# Autodesk Inventor assembly: caly_stół
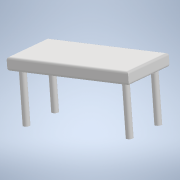
[picture p0: Inventor's stored thumbnail of the model, 180x180]
Saved by Autodesk Inventor 2021 (Build 250183000, 183)
## iProperties
Created: 2020-04-11
Part Number: caly_stół
Document SubType Name: Assembly
Designer: dyrag
Author: dyrag
## Documents named in this file (3)
- C:\Users\dyrag\Desktop\Projects\AutoCAD_Inventor_projects\stół\caly_stół.iam
- C:\Users\dyrag\Desktop\Projects\AutoCAD_Inventor_projects\stół\blat.ipt
- C:\Users\dyrag\Desktop\Projects\AutoCAD_Inventor_projects\stół\Noga.ipt
## Components (6 placed, 2 different names)
1. blat:1 — Zestawiające:1, Zestawiające:2, Zestawiające:3, Zestawiające:4, Równoległe:1, Równoległe:2, Zestawiające:5, Zestawiające:6, Zestawiające:7, Równoległe:3, Równoległe:4, Zestawiające:8, Równoległe:5, Równoległe:6, Zestawiające:9, Równoległe:7, Równoległe:8
2. Noga:1 — Zestawiające:4, Równoległe:1, Równoległe:2
3. Noga:2 — Zestawiające:5, Zestawiające:6
4. Noga:3 — Zestawiające:9, Równoległe:7, Równoległe:8
5. Noga:4 — Zestawiające:8, Równoległe:5, Równoległe:6
6. Noga:5 — Zestawiające:7, Równoległe:3, Równoległe:4
## Relationships (17: Mate 9, Flush 8)
- Zestawiające:1 [Mate]: blat:1
- Zestawiające:2 [Mate]: blat:1
- Zestawiające:3 [Mate]: blat:1
- Zestawiające:4 [Mate]: blat:1 ↔ Noga:1
- Równoległe:1 [Flush] (5 mm): blat:1 ↔ Noga:1
- Równoległe:2 [Flush] (5 mm): blat:1 ↔ Noga:1
- Zestawiające:5 [Mate]: blat:1 ↔ Noga:2
- Zestawiające:6 [Mate]: blat:1 ↔ Noga:2
- Zestawiające:7 [Mate]: blat:1 ↔ Noga:5
- Równoległe:3 [Flush] (-5 mm): blat:1 ↔ Noga:5
- Równoległe:4 [Flush] (-5 mm): blat:1 ↔ Noga:5
- Zestawiające:8 [Mate]: blat:1 ↔ Noga:4
- Równoległe:5 [Flush] (5 mm): blat:1 ↔ Noga:4
- Równoległe:6 [Flush] (5 mm): blat:1 ↔ Noga:4
- Zestawiające:9 [Mate]: blat:1 ↔ Noga:3
- Równoległe:7 [Flush] (5 mm): blat:1 ↔ Noga:3
- Równoległe:8 [Flush] (-5 mm): blat:1 ↔ Noga:3
